# Autodesk Inventor assembly: Stickman_FIght
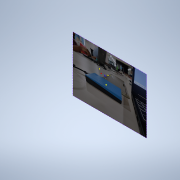
[picture p0: Inventor's stored thumbnail of the model, 180x180]
Saved by Autodesk Inventor 2022 (Build 260153000, 153)
## iProperties
Created: 2022-02-04
Part Number: Stickman_FIght
Document SubType Name: Assembly
Designer: joshw
Author: joshw
## Documents named in this file (5)
- D:\Fab_Labs\Week_3\Inventor_3D\Fun\Stickman_FIght.iam
- D:\Fab_Labs\Week_3\Inventor_3D\Fun\Body1.ipt
- D:\Fab_Labs\Week_3\Inventor_3D\Fun\body parts.ipt
- D:\Fab_Labs\Week_3\Inventor_3D\Fun\SXS.ipt
- D:\Fab_Labs\Week_3\Inventor_3D\Fun\gLOW_rED.ipt
## Components (23 placed, 4 different names)
1. Body1:1 — Rotational:1, Rotational:4, Rotational:6, Rotational:8
2. body parts:1 — Rotational:1, Rotational:2
3. body parts:2 — Rotational:2, Mate:5, Mate:6, Mate:7
4. body parts:4 — Mate:2, Mate:3, Mate:4
5. body parts:5 — Rotational:4
6. SXS:1 — Mate:1, Flush:3
7. body parts:6 — Rotational:6
8. body parts:7
9. body parts:8 — Rotational:8
10. body parts:9
11. Body1:2
12. body parts:10
13. body parts:11 — Mate:8, Mate:9, Mate:10
14. body parts:12 — Mate:11, Mate:12, Mate:13
15. body parts:13
16. body parts:14
17. body parts:15
18. body parts:16
19. body parts:17
20. gLOW_rED:1 — Mate:2, Mate:3, Mate:4
21. gLOW_rED:2 — Mate:5, Mate:6, Mate:7
22. gLOW_rED:3 — Mate:8, Mate:9, Mate:10
23. gLOW_rED:4 — Mate:11, Mate:12, Mate:13
## Relationships (30: RevoluteJoint 16, Mate 13, Flush 1)
- Rotational:1 [RevoluteJoint]: Body1:1 ↔ body parts:1
- Rotational:2 [RevoluteJoint]: body parts:1 ↔ body parts:2
- [RevoluteJoint]: body parts:4 ↔ body parts:5
- Rotational:4 [RevoluteJoint]: Body1:1 ↔ body parts:5
- Mate:1: SXS:1
- Flush:3: SXS:1
- [RevoluteJoint]: body parts:6 ↔ body parts:7
- Rotational:6 [RevoluteJoint]: Body1:1 ↔ body parts:6
- [RevoluteJoint]: body parts:8 ↔ body parts:9
- Rotational:8 [RevoluteJoint]: Body1:1 ↔ body parts:8
- [RevoluteJoint]: Body1:2 ↔ body parts:10
- [RevoluteJoint]: body parts:10 ↔ body parts:11
- [RevoluteJoint]: body parts:12 ↔ body parts:13
- [RevoluteJoint]: Body1:2 ↔ body parts:13
- [RevoluteJoint]: body parts:14 ↔ body parts:15
- [RevoluteJoint]: Body1:2 ↔ body parts:14
- [RevoluteJoint]: body parts:16 ↔ body parts:17
- [RevoluteJoint]: Body1:2 ↔ body parts:16
- Mate:2: body parts:4 ↔ gLOW_rED:1
- Mate:3: body parts:4 ↔ gLOW_rED:1
- Mate:4: body parts:4 ↔ gLOW_rED:1
- Mate:5: body parts:2 ↔ gLOW_rED:2
- Mate:6: body parts:2 ↔ gLOW_rED:2
- Mate:7: body parts:2 ↔ gLOW_rED:2
- Mate:8: body parts:11 ↔ gLOW_rED:3
- Mate:9: body parts:11 ↔ gLOW_rED:3
- Mate:10: body parts:11 ↔ gLOW_rED:3
- Mate:11: body parts:12 ↔ gLOW_rED:4
- Mate:12: body parts:12 ↔ gLOW_rED:4
- Mate:13: body parts:12 ↔ gLOW_rED:4
## Named parameters: d13_d11 = 0 mm, d14_d12 = 0.05942 deg, d19_d11 = 0 mm, d20_d12 = -47.773037 deg, d23_d19_d11 = 0 mm, d24_d20_d12 = -59.595436 deg, d27_d9 = 0 mm, d28_d10 = -43.77564 deg, d29_d11 = 0 mm, d30_d12 = -97.752849 deg, d31_d13_d11 = 0 mm, d32_d14_d12 = 160.558594 deg, d33_d15 = 0 mm, d34_d16 = 42.035706 deg, d35_d19_d11 = 0 mm, d36_d20_d12 = 36.694769 deg, d37_d21 = 0 mm, d38_d22 = 40.392132 deg, d39_d23_d19_d11 = 0 mm, d40_d24_d20_d12 = -1.282507 deg, d41_d25 = 0 mm, d42_d26 = 15.66296 deg
